# Autodesk Inventor assembly: uC
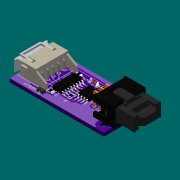
[picture p0: Inventor's stored thumbnail of the model, 180x180]
Saved by Autodesk Inventor 2016 (Build 200138000, 138)
## iProperties
Created: 2016-09-05
Part Number: uC
Document SubType Name: Assembly
Designer: sawaiz
Author: sawaiz
## Documents named in this file (13)
- C:\Users\sawaiz\oneDrive\projects\splitFlapDisplay\electronics\cad\uC\uC.iam
- C:\Users\sawaiz\oneDrive\projects\splitFlapDisplay\electronics\cad\component\SOT23.ipt
- C:\Users\sawaiz\oneDrive\projects\splitFlapDisplay\electronics\cad\component\chipResistor\chipResistor-0805.ipt
- C:\Users\sawaiz\oneDrive\projects\splitFlapDisplay\electronics\cad\component\chipResistor.ipt
- C:\Users\sawaiz\oneDrive\projects\splitFlapDisplay\electronics\cad\component\soic.ipt
- C:\Users\sawaiz\oneDrive\projects\splitFlapDisplay\electronics\cad\component\soic\soic-8-W.ipt
- C:\Users\sawaiz\oneDrive\projects\splitFlapDisplay\electronics\cad\component\soic\soic-16-N.ipt
- C:\Users\sawaiz\oneDrive\projects\splitFlapDisplay\electronics\cad\component\sod-80.ipt
- C:\Users\sawaiz\oneDrive\projects\splitFlapDisplay\electronics\cad\uC\uC.ipt
- C:\Users\sawaiz\oneDrive\projects\splitFlapDisplay\electronics\cad\component\XHP-5.ipt
- C:\Users\sawaiz\oneDrive\projects\splitFlapDisplay\electronics\cad\component\S5B-XH-A-1.ipt
- C:\Users\sawaiz\oneDrive\projects\splitFlapDisplay\electronics\cad\component\75867131lf\75867131lf.iam
- C:\Users\sawaiz\oneDrive\projects\splitFlapDisplay\electronics\cad\component\61200623021.ipt
## Components (14 placed, 10 different names)
1. SOT23:1 — Flush:7, Angle:17
2. chipResistor-0805:1 — Angle:5, Angle:12, Angle:13, Mate:2
3. chipResistor-0805:2 — Flush:2, Angle:15, Mate:1
4. chipResistor-0805:4 — Flush:1, Angle:5, Angle:6, Angle:7, Flush:11, Flush:12, Angle:13, Angle:14
5. chipResistor-0805:5 — Flush:1, Flush:2, Flush:5, Angle:6, Flush:8, Flush:9, Angle:12
6. chipResistor-0805:6 — Flush:5, Angle:7, Flush:10, Flush:11, Angle:16
7. soic-8-W:2 — Flush:6, Flush:7, Flush:8, Flush:12
8. soic-16-N:3 — Flush:6, Flush:9, Flush:10, Angle:14, Angle:15, Angle:16, Angle:17
9. sod-80:1 — Tangent:1, Angle:8
10. uC:1 — Tangent:1, Angle:8, Mate:1, Mate:2, Mate:3, Angle:18, Tangent:2, Angle:20
11. XHP-5:1 — Angle:19, Mate:4, Mate:5, Mate:6
12. S5B-XH-A-1:1 — Mate:3, Angle:18, Angle:19, Mate:4, Mate:5, Mate:6
13. 75867131lf:1 [sub-assembly] — Tangent:2, Angle:20, Mate:7, Mate:8
14. 61200623021:1 — Mate:7, Mate:8
## Relationships (33: Angle 13, Flush 10, Mate 8, Tangent 2)
- Flush:1: chipResistor-0805:4 ↔ chipResistor-0805:5
- Flush:2: chipResistor-0805:2 ↔ chipResistor-0805:5
- Flush:5: chipResistor-0805:5 ↔ chipResistor-0805:6
- Angle:5 (0 deg): chipResistor-0805:1 ↔ chipResistor-0805:4
- Angle:6 (0 deg): chipResistor-0805:4 ↔ chipResistor-0805:5
- Angle:7 (0 deg): chipResistor-0805:4 ↔ chipResistor-0805:6
- Flush:6: soic-8-W:2 ↔ soic-16-N:3
- Flush:7: SOT23:1 ↔ soic-8-W:2
- Flush:8: chipResistor-0805:5 ↔ soic-8-W:2
- Flush:9: chipResistor-0805:5 ↔ soic-16-N:3
- Flush:10: chipResistor-0805:6 ↔ soic-16-N:3
- Flush:11: chipResistor-0805:4 ↔ chipResistor-0805:6
- Flush:12: chipResistor-0805:4 ↔ soic-8-W:2
- Tangent:1: sod-80:1 ↔ uC:1
- Angle:8 (0 deg): sod-80:1 ↔ uC:1
- Angle:12 (0 deg): chipResistor-0805:1 ↔ chipResistor-0805:5
- Angle:13 (0 deg): chipResistor-0805:1 ↔ chipResistor-0805:4
- Angle:14 (0 deg): chipResistor-0805:4 ↔ soic-16-N:3
- Angle:15 (0 deg): chipResistor-0805:2 ↔ soic-16-N:3
- Angle:16 (0 deg): chipResistor-0805:6 ↔ soic-16-N:3
- Angle:17 (0 deg): SOT23:1 ↔ soic-16-N:3
- Mate:1: chipResistor-0805:2 ↔ uC:1
- Mate:2: chipResistor-0805:1 ↔ uC:1
- Mate:3: uC:1 ↔ S5B-XH-A-1:1
- Angle:18 (0 deg): uC:1 ↔ S5B-XH-A-1:1
- Angle:19 (0 deg): XHP-5:1 ↔ S5B-XH-A-1:1
- Mate:4: XHP-5:1 ↔ S5B-XH-A-1:1
- Mate:5: XHP-5:1 ↔ S5B-XH-A-1:1
- Mate:6: XHP-5:1 ↔ S5B-XH-A-1:1
- Tangent:2: uC:1 ↔ 75867131lf:1
- Angle:20 (0 deg): uC:1 ↔ 75867131lf:1
- Mate:7: 75867131lf:1 ↔ 61200623021:1
- Mate:8 (0.5 mm): 75867131lf:1 ↔ 61200623021:1
